# Autodesk Inventor assembly: RT_ELE_A_006_ESTOP
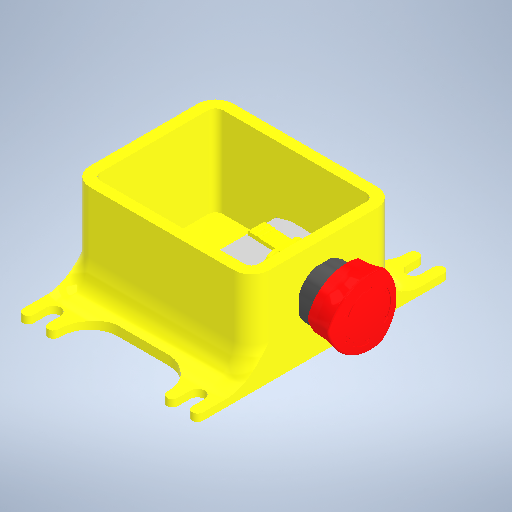
[picture p0: Inventor's stored thumbnail of the model, 512x512]
Saved by Autodesk Inventor 2025.3 (Build 293356000, 356)
## iProperties
Created: 2026-06-07
Part Number: RT_ELE_A_006_ESTOP
Document SubType Name: Assembly
Designer: louis
Author: louis
## Documents named in this file (3)
- C:\Users\louis\OneDrive\Desktop\R_Trident\02_CAD\04_Subassemblies\RT_ELE_A_006_ESTOP.iam
- C:\Users\louis\OneDrive\Desktop\R_Trident\02_CAD\03_Parts_Custom\RT_ELE_PR_016_ESTOP_Enclosure.ipt
- C:\Users\louis\OneDrive\Desktop\R_Trident\02_CAD\01_Standard_Parts\04_ELE_Electrical_Automation\L22ED01D\L22ED01D.iam
## Components (2 placed, 2 different names)
1. RT_ELE_PR_016_ESTOP_Enclosure:1 — Mate:1, Mate:2, Mate:3, Mate:4, Flush:6
2. L22ED01D:1 [sub-assembly] — Mate:3, Mate:4, Flush:6
## Relationships (5: Mate 4, Flush 1)
- Mate:1: RT_ELE_PR_016_ESTOP_Enclosure:1
- Mate:2: RT_ELE_PR_016_ESTOP_Enclosure:1
- Mate:3: RT_ELE_PR_016_ESTOP_Enclosure:1 ↔ L22ED01D:1
- Mate:4: RT_ELE_PR_016_ESTOP_Enclosure:1 ↔ L22ED01D:1
- Flush:6: RT_ELE_PR_016_ESTOP_Enclosure:1 ↔ L22ED01D:1
